# Autodesk Inventor assembly: Montagem do Conjunto de Engrenagens
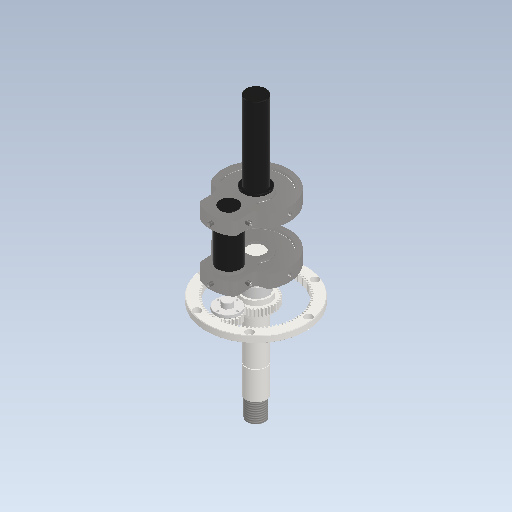
[picture p0: Inventor's stored thumbnail of the model, 512x512]
Saved by Autodesk Inventor 2021 (Build 250183000, 183)
## iProperties
Category: 10
Company: UFABC
Created: 2021-07-26
Document SubType Name: Assembly
Designer: Giovanni
Checked By: Prof. Luis
User Status: 1:4
Author: Giovanni
Title: Montagem do Conjunto de Engrenagens
Keywords: 6
## Documents named in this file (10)
- C:\Users\irineu\Documents\Inventor\MotorRadial7\Conjunto de Engrenagens.iam
- C:\Users\irineu\Documents\Inventor\MotorRadial7\Conjunto_Virabrequim.iam
- C:\Users\irineu\Documents\Inventor\Content Center Files\R2021\pt-BR\DIN 6885-1 A\DIN 6885 - A 12 x 8 x 32.ipt
- C:\Users\irineu\Documents\Inventor\MotorRadial7\Engrenagens.iam
- C:\Users\irineu\Documents\Inventor\MotorRadial7\Peça42.ipt
- C:\Users\irineu\Documents\Inventor\MotorRadial7\Peça41.ipt
- C:\Users\irineu\Documents\Inventor\MotorRadial7\Engrenagens 2.iam
- C:\Users\irineu\Documents\Inventor\MotorRadial7\Engrenagens 3.iam
- C:\Users\irineu\Documents\Inventor\MotorRadial7\Peça43.ipt
- C:\Users\irineu\Documents\Inventor\Content Center Files\R2021\pt-BR\DIN 471(1)\DIN 471 - 21x1,2.ipt
## Components (9 placed, 9 different names)
1. Conjunto_Virabrequim:1 [sub-assembly] — Coincidente:1, Coincidente:2, Coincidente:3, Coincidente:4, Coincidente:5, Coincidente:6, Coincidente:8, Coincidente:11
2. DIN 6885-1 A A 12 x 8 x 32:1 — Coincidente:3, Coincidente:4, Coincidente:5, Coincidente:7
3. Engrenagens:1 [sub-assembly] — Coincidente:6, Coincidente:7, Inserir:1, Coincidente:10, Rotação:1
4. Peça42:1 — Inserir:1, Coincidente:8
5. Peça41:1 — Coincidente:9, Alinhado:1, Coincidente:10, Inserir:2
6. Engrenagens 2:1 [sub-assembly] — Inserir:2, Rotação:1, Alinhado:2, Rotação:2, Inserir:3, Alinhado:3
7. Engrenagens 3:1 [sub-assembly] — Coincidente:11, Alinhado:2, Rotação:2
8. Peça43:1 — Inserir:3, Inserir:4
9. DIN 471 21x1,2:1 — Inserir:4, Alinhado:3
## Relationships (20: Mate 11, Insert 4, Flush 3, RelateRotation 2)
- Coincidente:1 [Mate]: Conjunto_Virabrequim:1
- Coincidente:2 [Mate]: Conjunto_Virabrequim:1
- Coincidente:3 [Mate]: Conjunto_Virabrequim:1 ↔ DIN 6885-1 A A 12 x 8 x 32:1
- Coincidente:4 [Mate]: Conjunto_Virabrequim:1 ↔ DIN 6885-1 A A 12 x 8 x 32:1
- Coincidente:5 [Mate]: Conjunto_Virabrequim:1 ↔ DIN 6885-1 A A 12 x 8 x 32:1
- Coincidente:6 [Mate]: Conjunto_Virabrequim:1 ↔ Engrenagens:1
- Coincidente:7 [Mate]: DIN 6885-1 A A 12 x 8 x 32:1 ↔ Engrenagens:1
- Inserir:1: Engrenagens:1 ↔ Peça42:1
- Coincidente:8 [Mate] (15 mm): Conjunto_Virabrequim:1 ↔ Peça42:1
- Coincidente:9 [Mate]: Peça41:1
- Alinhado:1 [Flush] (-56 mm): Peça41:1
- Coincidente:10 [Mate]: Engrenagens:1 ↔ Peça41:1
- Inserir:2: Peça41:1 ↔ Engrenagens 2:1
- Rotação:1 [RelateRotation] (1.56 ul): Engrenagens:1 ↔ Engrenagens 2:1
- Coincidente:11 [Mate]: Conjunto_Virabrequim:1 ↔ Engrenagens 3:1
- Alinhado:2 [Flush]: Engrenagens 2:1 ↔ Engrenagens 3:1
- Rotação:2 [RelateRotation] (0.2809 ul): Engrenagens 2:1 ↔ Engrenagens 3:1
- Inserir:3: Engrenagens 2:1 ↔ Peça43:1
- Inserir:4: Peça43:1 ↔ DIN 471 21x1,2:1
- Alinhado:3 [Flush]: Engrenagens 2:1 ↔ DIN 471 21x1,2:1
